# Autodesk Inventor assembly: Radius Gauge
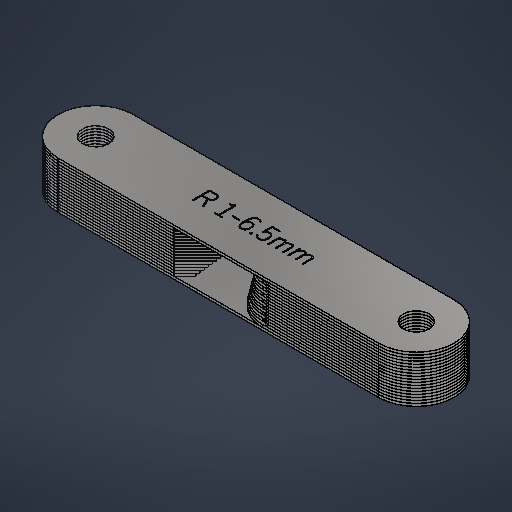
[picture p0: Inventor's stored thumbnail of the model, 512x512]
Saved by Autodesk Inventor 2026 (Build 300175050, 175E)
## iProperties
Created: 2025-07-21
Part Number: Radius Gauge
Document SubType Name: Assembly
Designer: Joshua Eah
Author: Joshua Eah
## Documents named in this file (35)
- C:\Users\Joshua Eah\Documents\GitHub\DesignedTrinkets\Radius Gauge\Radius Gauge.iam
- C:\Users\Joshua Eah\Documents\GitHub\DesignedTrinkets\Radius Gauge\Bottom Case.ipt
- C:\Users\Joshua Eah\Documents\GitHub\DesignedTrinkets\Radius Gauge\Internal Radius Gauge\6mm.ipt
- C:\Users\Joshua Eah\Documents\GitHub\DesignedTrinkets\Radius Gauge\Internal Radius Gauge\1.5mm.ipt
- C:\Users\Joshua Eah\Documents\GitHub\DesignedTrinkets\Radius Gauge\Internal Radius Gauge\1.25mm.ipt
- C:\Users\Joshua Eah\Documents\GitHub\DesignedTrinkets\Radius Gauge\Internal Radius Gauge\1.75mm.ipt
- C:\Users\Joshua Eah\Documents\GitHub\DesignedTrinkets\Radius Gauge\Internal Radius Gauge\1mm.ipt
- C:\Users\Joshua Eah\Documents\GitHub\DesignedTrinkets\Radius Gauge\Internal Radius Gauge\2.5mm.ipt
- C:\Users\Joshua Eah\Documents\GitHub\DesignedTrinkets\Radius Gauge\Internal Radius Gauge\2mm.ipt
- C:\Users\Joshua Eah\Documents\GitHub\DesignedTrinkets\Radius Gauge\Internal Radius Gauge\3.5mm.ipt
- C:\Users\Joshua Eah\Documents\GitHub\DesignedTrinkets\Radius Gauge\Internal Radius Gauge\3mm.ipt
- C:\Users\Joshua Eah\Documents\GitHub\DesignedTrinkets\Radius Gauge\Internal Radius Gauge\4.5mm.ipt
- C:\Users\Joshua Eah\Documents\GitHub\DesignedTrinkets\Radius Gauge\Internal Radius Gauge\4mm.ipt
- C:\Users\Joshua Eah\Documents\GitHub\DesignedTrinkets\Radius Gauge\Internal Radius Gauge\5.5mm.ipt
- C:\Users\Joshua Eah\Documents\GitHub\DesignedTrinkets\Radius Gauge\Internal Radius Gauge\5mm.ipt
- C:\Users\Joshua Eah\Documents\GitHub\DesignedTrinkets\Radius Gauge\Internal Radius Gauge\6.5mm.ipt
- C:\Users\Joshua Eah\Documents\GitHub\DesignedTrinkets\Radius Gauge\Internal Radius Gauge\2.25mm.ipt
- C:\Users\Joshua Eah\Documents\GitHub\DesignedTrinkets\Radius Gauge\Internal Radius Gauge\2.75mm.ipt
- C:\Users\Joshua Eah\Documents\GitHub\DesignedTrinkets\Radius Gauge\External Radius Gauge\E5mm.ipt
- C:\Users\Joshua Eah\Documents\GitHub\DesignedTrinkets\Radius Gauge\External Radius Gauge\E6.5mm.ipt
- C:\Users\Joshua Eah\Documents\GitHub\DesignedTrinkets\Radius Gauge\External Radius Gauge\E6mm.ipt
- C:\Users\Joshua Eah\Documents\GitHub\DesignedTrinkets\Radius Gauge\External Radius Gauge\E5.5mm.ipt
- C:\Users\Joshua Eah\Documents\GitHub\DesignedTrinkets\Radius Gauge\External Radius Gauge\E4.5mm.ipt
- C:\Users\Joshua Eah\Documents\GitHub\DesignedTrinkets\Radius Gauge\External Radius Gauge\E4mm.ipt
- C:\Users\Joshua Eah\Documents\GitHub\DesignedTrinkets\Radius Gauge\External Radius Gauge\E3.5mm.ipt
- C:\Users\Joshua Eah\Documents\GitHub\DesignedTrinkets\Radius Gauge\External Radius Gauge\E3mm.ipt
- C:\Users\Joshua Eah\Documents\GitHub\DesignedTrinkets\Radius Gauge\External Radius Gauge\E2.75mm.ipt
- C:\Users\Joshua Eah\Documents\GitHub\DesignedTrinkets\Radius Gauge\External Radius Gauge\E2mm.ipt
- C:\Users\Joshua Eah\Documents\GitHub\DesignedTrinkets\Radius Gauge\External Radius Gauge\E2.5mm.ipt
- C:\Users\Joshua Eah\Documents\GitHub\DesignedTrinkets\Radius Gauge\External Radius Gauge\E2.25mm.ipt
- C:\Users\Joshua Eah\Documents\GitHub\DesignedTrinkets\Radius Gauge\External Radius Gauge\E1.5mm.ipt
- C:\Users\Joshua Eah\Documents\GitHub\DesignedTrinkets\Radius Gauge\External Radius Gauge\E1.25mm.ipt
- C:\Users\Joshua Eah\Documents\GitHub\DesignedTrinkets\Radius Gauge\External Radius Gauge\E1.75mm.ipt
- C:\Users\Joshua Eah\Documents\GitHub\DesignedTrinkets\Radius Gauge\External Radius Gauge\E1mm.ipt
- C:\Users\Joshua Eah\Documents\GitHub\DesignedTrinkets\Radius Gauge\Top Case.ipt
## Components (34 placed, 34 different names)
1. Bottom Case:1 — Rotational:1, Rotational:17
2. 6.5mm:1 — Rotational:1, Rotational:2
3. 6mm:1 — Rotational:2, Rotational:3
4. 4.5mm:1 — Rotational:5, Rotational:6
5. 4mm:1 — Rotational:6, Rotational:7
6. 5.5mm:1 — Rotational:3, Rotational:4
7. 5mm:1 — Rotational:4, Rotational:5
8. 1.5mm:1 — Rotational:14, Rotational:15
9. 1.25mm:1 — Rotational:15, Rotational:16
10. 1.75mm:1 — Rotational:13, Rotational:14
11. 1mm:1 — Rotational:16, Rotational:34
12. 2.5mm:1 — Rotational:10, Rotational:11
13. 2.25mm:1 — Rotational:11, Rotational:12
14. 2.75mm:1 — Rotational:9, Rotational:10
15. 2mm:1 — Rotational:12, Rotational:13
16. 3.5mm:1 — Rotational:7, Rotational:8
17. 3mm:1 — Rotational:8, Rotational:9
18. E5mm:1 — Rotational:20, Rotational:21
19. E6.5mm:1 — Rotational:17, Rotational:18
20. E6mm:1 — Rotational:18, Rotational:19
21. E5.5mm:1 — Rotational:19, Rotational:20
22. E4.5mm:1 — Rotational:21, Rotational:22
23. E4mm:1 — Rotational:22, Rotational:23
24. E3.5mm:1 — Rotational:23, Rotational:24
25. E3mm:1 — Rotational:24, Rotational:25
26. E2.75mm:1 — Rotational:25, Rotational:26
27. E2mm:1 — Rotational:28, Rotational:29
28. E2.5mm:1 — Rotational:26, Rotational:27
29. E2.25mm:1 — Rotational:27, Rotational:28
30. E1.5mm:1 — Rotational:30, Rotational:31
31. E1.25mm:1 — Rotational:31, Rotational:32
32. E1.75mm:1 — Rotational:29, Rotational:30
33. E1mm:1 — Rotational:32, Rotational:33
34. Top Case:1 — Rotational:33, Rotational:34
## Relationships (34: RevoluteJoint 34)
- Rotational:1 [RevoluteJoint]: Bottom Case:1 ↔ 6.5mm:1
- Rotational:2 [RevoluteJoint]: 6.5mm:1 ↔ 6mm:1
- Rotational:3 [RevoluteJoint]: 6mm:1 ↔ 5.5mm:1
- Rotational:4 [RevoluteJoint]: 5.5mm:1 ↔ 5mm:1
- Rotational:5 [RevoluteJoint]: 4.5mm:1 ↔ 5mm:1
- Rotational:6 [RevoluteJoint]: 4.5mm:1 ↔ 4mm:1
- Rotational:7 [RevoluteJoint]: 4mm:1 ↔ 3.5mm:1
- Rotational:8 [RevoluteJoint]: 3.5mm:1 ↔ 3mm:1
- Rotational:9 [RevoluteJoint]: 2.75mm:1 ↔ 3mm:1
- Rotational:10 [RevoluteJoint]: 2.5mm:1 ↔ 2.75mm:1
- Rotational:11 [RevoluteJoint]: 2.5mm:1 ↔ 2.25mm:1
- Rotational:12 [RevoluteJoint]: 2.25mm:1 ↔ 2mm:1
- Rotational:13 [RevoluteJoint]: 1.75mm:1 ↔ 2mm:1
- Rotational:14 [RevoluteJoint]: 1.5mm:1 ↔ 1.75mm:1
- Rotational:15 [RevoluteJoint]: 1.5mm:1 ↔ 1.25mm:1
- Rotational:16 [RevoluteJoint]: 1.25mm:1 ↔ 1mm:1
- Rotational:17 [RevoluteJoint]: Bottom Case:1 ↔ E6.5mm:1
- Rotational:18 [RevoluteJoint]: E6.5mm:1 ↔ E6mm:1
- Rotational:19 [RevoluteJoint]: E6mm:1 ↔ E5.5mm:1
- Rotational:20 [RevoluteJoint]: E5mm:1 ↔ E5.5mm:1
- Rotational:21 [RevoluteJoint]: E5mm:1 ↔ E4.5mm:1
- Rotational:22 [RevoluteJoint]: E4.5mm:1 ↔ E4mm:1
- Rotational:23 [RevoluteJoint]: E4mm:1 ↔ E3.5mm:1
- Rotational:24 [RevoluteJoint]: E3.5mm:1 ↔ E3mm:1
- Rotational:25 [RevoluteJoint]: E3mm:1 ↔ E2.75mm:1
- Rotational:26 [RevoluteJoint]: E2.75mm:1 ↔ E2.5mm:1
- Rotational:27 [RevoluteJoint]: E2.5mm:1 ↔ E2.25mm:1
- Rotational:28 [RevoluteJoint]: E2mm:1 ↔ E2.25mm:1
- Rotational:29 [RevoluteJoint]: E2mm:1 ↔ E1.75mm:1
- Rotational:30 [RevoluteJoint]: E1.5mm:1 ↔ E1.75mm:1
- Rotational:31 [RevoluteJoint]: E1.5mm:1 ↔ E1.25mm:1
- Rotational:32 [RevoluteJoint]: E1.25mm:1 ↔ E1mm:1
- Rotational:33 [RevoluteJoint]: E1mm:1 ↔ Top Case:1
- Rotational:34 [RevoluteJoint]: 1mm:1 ↔ Top Case:1
